# Autodesk Inventor assembly: Ares
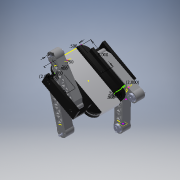
[picture p0: Inventor's stored thumbnail of the model, 180x180]
Saved by Autodesk Inventor 2018.2 (Build 222227000, 227)
## iProperties
Created: 2018-02-01
Part Number: Ares
Document SubType Name: Assembly
Designer: MIABo
Author: MIABo
## Documents named in this file (5)
- C:\Users\MIABo\OneDrive\Documents\GitHub\Ares\Ares.iam
- C:\Users\MIABo\OneDrive\Documents\GitHub\Ares\SUspension mounting.ipt
- C:\Users\MIABo\OneDrive\Documents\GitHub\Ares\Frame.ipt
- C:\Users\MIABo\OneDrive\Documents\GitHub\Ares\Leg Assembly.ipt
- C:\Users\MIABo\OneDrive\Documents\GitHub\Ares\wheel motor.ipt
## Components (11 placed, 4 different names)
1. SUspension mounting:1 — Mate:1, Mate:2, Mate:3, Mate:7, Rotational:1, Rotational:2
2. Frame:1 — Mate:1, Mate:2, Mate:3, Mate:4, Mate:5, Mate:6, Mate:7
3. SUspension mounting:2 — Mate:4, Mate:5, Mate:6, Rotational:3, Rotational:4
4. Leg Assembly:1 — Rotational:4, Mate:11, Mate:12, Mate:13, Mate:14
5. Leg Assembly:2 — Rotational:2, Mate:18, Mate:19, Mate:20
6. Leg Assembly:3 — Rotational:1, Mate:15, Mate:16, Mate:17
7. Leg Assembly:4 — Rotational:3, Mate:8, Mate:9, Mate:10
8. wheel motor:1 — Mate:18, Mate:19, Mate:20
9. wheel motor:2 — Mate:15, Mate:16, Mate:17
10. wheel motor:3 — Mate:8, Mate:9, Mate:10
11. wheel motor:4 — Mate:11, Mate:12, Mate:13, Mate:14
## Relationships (24: Mate 20, RevoluteJoint 4)
- Mate:1: SUspension mounting:1 ↔ Frame:1
- Mate:2: SUspension mounting:1 ↔ Frame:1
- Mate:3: SUspension mounting:1 ↔ Frame:1
- Mate:4: Frame:1 ↔ SUspension mounting:2
- Mate:5: Frame:1 ↔ SUspension mounting:2
- Mate:6: Frame:1 ↔ SUspension mounting:2
- Mate:7: SUspension mounting:1 ↔ Frame:1
- Rotational:1 [RevoluteJoint]: SUspension mounting:1 ↔ Leg Assembly:3
- Rotational:2 [RevoluteJoint]: SUspension mounting:1 ↔ Leg Assembly:2
- Rotational:3 [RevoluteJoint] (1.27 mm): SUspension mounting:2 ↔ Leg Assembly:4
- Rotational:4 [RevoluteJoint] (1.27 mm): SUspension mounting:2 ↔ Leg Assembly:1
- Mate:8: Leg Assembly:4 ↔ wheel motor:3
- Mate:9: Leg Assembly:4 ↔ wheel motor:3
- Mate:10: Leg Assembly:4 ↔ wheel motor:3
- Mate:11: Leg Assembly:1 ↔ wheel motor:4
- Mate:12: Leg Assembly:1 ↔ wheel motor:4
- Mate:13: Leg Assembly:1 ↔ wheel motor:4
- Mate:14: Leg Assembly:1 ↔ wheel motor:4
- Mate:15: Leg Assembly:3 ↔ wheel motor:2
- Mate:16: Leg Assembly:3 ↔ wheel motor:2
- Mate:17: Leg Assembly:3 ↔ wheel motor:2
- Mate:18: Leg Assembly:2 ↔ wheel motor:1
- Mate:19: Leg Assembly:2 ↔ wheel motor:1
- Mate:20: Leg Assembly:2 ↔ wheel motor:1
